# Autodesk Inventor assembly: lp-box
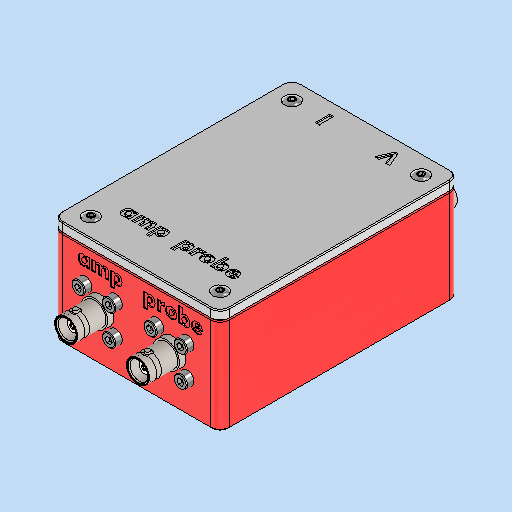
[picture p0: Inventor's stored thumbnail of the model, 512x512]
Saved by Autodesk Inventor 2025 (Build 290162000, 162)
## iProperties
Created: 2024-12-23
Part Number: lp-box
Document SubType Name: Assembly
Designer: kuzmin
Author: kuzmin
## Documents named in this file (9)
- C:\Users\queez\Dropbox\Drawings\PIHTI\ElectronicsBox\lp-box.iam
- C:\Users\queez\Dropbox\Drawings\PIHTI\ElectronicsBox\lp-box.ipt
- C:\Users\queez\Dropbox\Drawings\PIHTI\ContentCenter\Electrics\Amphenol RF 31-203-RFX v1\Amphenol RF 31-203-RFX v1.ipt
- C:\Users\queez\Dropbox\Drawings\PIHTI\ContentCenter\Fastners\M3x8-SHCS.ipt
- C:\Users\queez\Dropbox\Drawings\PIHTI\ElectronicsBox\bnc-nut-holder.iam
- C:\Users\queez\Dropbox\Drawings\PIHTI\ElectronicsBox\lp-box-lid.ipt
- C:\Users\queez\Dropbox\Drawings\PIHTI\ContentCenter\Fastners\M3x8-BHCS.ipt
- C:\Users\queez\Dropbox\Drawings\PIHTI\ContentCenter\Fastners\brass-insert-m3x5.ipt
- C:\Users\queez\Dropbox\Drawings\PIHTI\ElectronicsBox\firstki\firstki.iam
## Components (43 placed, 8 different names)
1. lp-box:1 — Rotational:1, Rotational:2, Rotational:3, Rotational:4, Rigid:9, Rigid:10, Rigid:11, Rigid:12, Rigid:13, Rigid:14, Rigid:15, Rigid:16, Rigid:20, Rotational:8, Rigid:23, Rigid:24, Rigid:25, Rigid:26, Rigid:27, Rigid:28, Rigid:29, Rigid:30, Rigid:31, Rigid:32, Rigid:33, Rigid:34, Rigid:35, Rigid:36, Rigid:37, Rigid:38
2. Amphenol RF 31-203-RFX v1:1 — Rotational:1, Rotational:5
3. Amphenol RF 31-203-RFX v1:2 — Rotational:4, Rigid:17
4. Amphenol RF 31-203-RFX v1:3 — Rotational:2, Rigid:18
5. Amphenol RF 31-203-RFX v1:4 — Rotational:3, Rigid:19
6. lp-box-lid:1 — Rigid:20, Rigid:21, Rigid:22, Rotational:6, Rotational:7
7. firstki:1 [sub-assembly] — Rigid:38
8. SS ISO 4762 M3 x 8:17
9. SS ISO 4762 M3 x 8:18
10. SS ISO 4762 M3 x 8:19
11. SS ISO 4762 M3 x 8:20
12. brass-insert-m3x5:1 — Rigid:31
13. brass-insert-m3x5:2 — Rigid:30
14. brass-insert-m3x5:3 — Rigid:32
15. brass-insert-m3x5:4 — Rigid:34
16. brass-insert-m3x5:5 — Rigid:35
17. brass-insert-m3x5:6 — Rigid:33
18. brass-insert-m3x5:7 — Rigid:37
19. brass-insert-m3x5:8 — Rigid:36
20. BS 4168 : Part 6 Hexagon socket countersunk and button head screws - Metric series - Metric M3 x 8:9 — Rigid:26
21. BS 4168 : Part 6 Hexagon socket countersunk and button head screws - Metric series - Metric M3 x 8:10 — Rigid:27
22. BS 4168 : Part 6 Hexagon socket countersunk and button head screws - Metric series - Metric M3 x 8:11 — Rigid:28
23. BS 4168 : Part 6 Hexagon socket countersunk and button head screws - Metric series - Metric M3 x 8:12 — Rigid:29
24. bnc-nut-holder:1 [sub-assembly] — Rotational:5
25. bnc-nut-holder:2 [sub-assembly] — Rigid:18
26. bnc-nut-holder:3 [sub-assembly] — Rigid:19
27. bnc-nut-holder:4 [sub-assembly] — Rigid:17
28. BS 4168 : Part 6 Hexagon socket countersunk and button head screws - Metric series - Metric M3 x 8:1 — Rotational:7
29. BS 4168 : Part 6 Hexagon socket countersunk and button head screws - Metric series - Metric M3 x 8:2 — Rigid:22
30. BS 4168 : Part 6 Hexagon socket countersunk and button head screws - Metric series - Metric M3 x 8:3 — Rotational:6
31. BS 4168 : Part 6 Hexagon socket countersunk and button head screws - Metric series - Metric M3 x 8:4 — Rigid:21
32. BS 4168 : Part 6 Hexagon socket countersunk and button head screws - Metric series - Metric M3 x 8:5 — Rotational:8
33. BS 4168 : Part 6 Hexagon socket countersunk and button head screws - Metric series - Metric M3 x 8:6 — Rigid:23
34. BS 4168 : Part 6 Hexagon socket countersunk and button head screws - Metric series - Metric M3 x 8:7 — Rigid:24
35. BS 4168 : Part 6 Hexagon socket countersunk and button head screws - Metric series - Metric M3 x 8:8 — Rigid:25
36. SS ISO 4762 M3 x 8:9 — Rigid:15
37. SS ISO 4762 M3 x 8:10 — Rigid:16
38. SS ISO 4762 M3 x 8:11 — Rigid:14
39. SS ISO 4762 M3 x 8:12 — Rigid:13
40. SS ISO 4762 M3 x 8:13 — Rigid:11
41. SS ISO 4762 M3 x 8:14 — Rigid:10
42. SS ISO 4762 M3 x 8:15 — Rigid:12
43. SS ISO 4762 M3 x 8:16 — Rigid:9
## Relationships (38: WeldJoint 30, RevoluteJoint 8)
- Rotational:1 [RevoluteJoint]: lp-box:1 ↔ Amphenol RF 31-203-RFX v1:1
- Rotational:2 [RevoluteJoint]: lp-box:1 ↔ Amphenol RF 31-203-RFX v1:3
- Rotational:3 [RevoluteJoint]: lp-box:1 ↔ Amphenol RF 31-203-RFX v1:4
- Rotational:4 [RevoluteJoint]: lp-box:1 ↔ Amphenol RF 31-203-RFX v1:2
- Rigid:9 [WeldJoint]: lp-box:1 ↔ SS ISO 4762 M3 x 8:16
- Rigid:10 [WeldJoint]: lp-box:1 ↔ SS ISO 4762 M3 x 8:14
- Rigid:11 [WeldJoint]: lp-box:1 ↔ SS ISO 4762 M3 x 8:13
- Rigid:12 [WeldJoint]: lp-box:1 ↔ SS ISO 4762 M3 x 8:15
- Rigid:13 [WeldJoint]: lp-box:1 ↔ SS ISO 4762 M3 x 8:12
- Rigid:14 [WeldJoint]: lp-box:1 ↔ SS ISO 4762 M3 x 8:11
- Rigid:15 [WeldJoint]: lp-box:1 ↔ SS ISO 4762 M3 x 8:9
- Rigid:16 [WeldJoint]: lp-box:1 ↔ SS ISO 4762 M3 x 8:10
- Rotational:5 [RevoluteJoint]: Amphenol RF 31-203-RFX v1:1 ↔ bnc-nut-holder:1
- Rigid:17 [WeldJoint]: Amphenol RF 31-203-RFX v1:2 ↔ bnc-nut-holder:4
- Rigid:18 [WeldJoint]: Amphenol RF 31-203-RFX v1:3 ↔ bnc-nut-holder:2
- Rigid:19 [WeldJoint]: Amphenol RF 31-203-RFX v1:4 ↔ bnc-nut-holder:3
- Rigid:20 [WeldJoint]: lp-box:1 ↔ lp-box-lid:1
- Rigid:21 [WeldJoint] (0.8 mm): lp-box-lid:1 ↔ BS 4168 : Part 6 Hexagon socket countersunk and button head screws - Metric series - Metric M3 x 8:4
- Rigid:22 [WeldJoint] (0.8 mm): lp-box-lid:1 ↔ BS 4168 : Part 6 Hexagon socket countersunk and button head screws - Metric series - Metric M3 x 8:2
- Rotational:6 [RevoluteJoint] (0.8 mm): lp-box-lid:1 ↔ BS 4168 : Part 6 Hexagon socket countersunk and button head screws - Metric series - Metric M3 x 8:3
- Rotational:7 [RevoluteJoint] (0.8 mm): lp-box-lid:1 ↔ BS 4168 : Part 6 Hexagon socket countersunk and button head screws - Metric series - Metric M3 x 8:1
- Rotational:8 [RevoluteJoint]: lp-box:1 ↔ BS 4168 : Part 6 Hexagon socket countersunk and button head screws - Metric series - Metric M3 x 8:5
- Rigid:23 [WeldJoint]: lp-box:1 ↔ BS 4168 : Part 6 Hexagon socket countersunk and button head screws - Metric series - Metric M3 x 8:6
- Rigid:24 [WeldJoint]: lp-box:1 ↔ BS 4168 : Part 6 Hexagon socket countersunk and button head screws - Metric series - Metric M3 x 8:7
- Rigid:25 [WeldJoint]: lp-box:1 ↔ BS 4168 : Part 6 Hexagon socket countersunk and button head screws - Metric series - Metric M3 x 8:8
- Rigid:26 [WeldJoint]: lp-box:1 ↔ BS 4168 : Part 6 Hexagon socket countersunk and button head screws - Metric series - Metric M3 x 8:9
- Rigid:27 [WeldJoint]: lp-box:1 ↔ BS 4168 : Part 6 Hexagon socket countersunk and button head screws - Metric series - Metric M3 x 8:10
- Rigid:28 [WeldJoint]: lp-box:1 ↔ BS 4168 : Part 6 Hexagon socket countersunk and button head screws - Metric series - Metric M3 x 8:11
- Rigid:29 [WeldJoint]: lp-box:1 ↔ BS 4168 : Part 6 Hexagon socket countersunk and button head screws - Metric series - Metric M3 x 8:12
- Rigid:30 [WeldJoint]: lp-box:1 ↔ brass-insert-m3x5:2
- Rigid:31 [WeldJoint]: lp-box:1 ↔ brass-insert-m3x5:1
- Rigid:32 [WeldJoint]: lp-box:1 ↔ brass-insert-m3x5:3
- Rigid:33 [WeldJoint]: lp-box:1 ↔ brass-insert-m3x5:6
- Rigid:34 [WeldJoint]: lp-box:1 ↔ brass-insert-m3x5:4
- Rigid:35 [WeldJoint]: lp-box:1 ↔ brass-insert-m3x5:5
- Rigid:36 [WeldJoint]: lp-box:1 ↔ brass-insert-m3x5:8
- Rigid:37 [WeldJoint]: lp-box:1 ↔ brass-insert-m3x5:7
- Rigid:38 [WeldJoint]: lp-box:1 ↔ firstki:1
